# Autodesk Inventor assembly: Enclosure Assembly
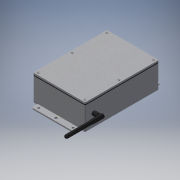
[picture p0: Inventor's stored thumbnail of the model, 180x180]
Saved by Autodesk Inventor 2019 (Build 230136000, 136)
## iProperties
Created: 2020-02-21
Part Number: Enclosure Assembly
Document SubType Name: Assembly
Designer: ntb11189
Author: ntb11189
## Documents named in this file (7)
- N:\Sandpit\Callum Brooksby\Main Enclosure\Enclosure Assembly.iam
- N:\Sandpit\Callum Brooksby\Main Enclosure\Main Enclosure Base.ipt
- N:\Sandpit\Callum Brooksby\Main Enclosure\gasket.ipt
- N:\Sandpit\Callum Brooksby\Main Enclosure\lid.ipt
- N:\Sandpit\Callum Brooksby\Main Enclosure\Antenna\Antenna.iam
- N:\Sandpit\Callum Brooksby\Main Enclosure\panel-connector\DBConnector-INV\Dsub 9 Pin, 2 Row, Female.ipt
- N:\Sandpit\Callum Brooksby\Main Enclosure\pj-005a.ipt
## Components (6 placed, 6 different names)
1. Main Enclosure Base:1 — Mate:2, Flush:3, Flush:4, Mate:3, Mate:4, Flush:5, Insert:1, Mate:5, Tangent:1, Tangent:2, Mate:6, Insert:2
2. gasket:1 — Mate:1, Flush:1, Flush:2, Mate:2
3. lid:1 — Mate:1, Flush:1, Flush:2, Flush:3, Flush:4
4. Antenna:1 [sub-assembly] — Insert:1, Angle:1
5. Dsub 9 Pin, 2 Row, Female:1 — Mate:5, Tangent:1, Tangent:2, Mate:6
6. pj-005a:1 — Insert:2
## Relationships (16: Mate 6, Flush 5, Insert 2, Tangent 2, Angle 1)
- Mate:1: gasket:1 ↔ lid:1
- Flush:1: gasket:1 ↔ lid:1
- Flush:2: gasket:1 ↔ lid:1
- Mate:2: Main Enclosure Base:1 ↔ gasket:1
- Flush:3: Main Enclosure Base:1 ↔ lid:1
- Flush:4: Main Enclosure Base:1 ↔ lid:1
- Mate:3 (-53 mm): Main Enclosure Base:1
- Mate:4: Main Enclosure Base:1
- Flush:5: Main Enclosure Base:1
- Insert:1: Main Enclosure Base:1 ↔ Antenna:1
- Angle:1 (180 deg): Antenna:1
- Mate:5: Main Enclosure Base:1 ↔ Dsub 9 Pin, 2 Row, Female:1
- Tangent:1: Main Enclosure Base:1 ↔ Dsub 9 Pin, 2 Row, Female:1
- Tangent:2: Main Enclosure Base:1 ↔ Dsub 9 Pin, 2 Row, Female:1
- Mate:6 (1.5 mm): Main Enclosure Base:1 ↔ Dsub 9 Pin, 2 Row, Female:1
- Insert:2: Main Enclosure Base:1 ↔ pj-005a:1
